# Autodesk Inventor assembly: ASY NDM_VOS pillar 1
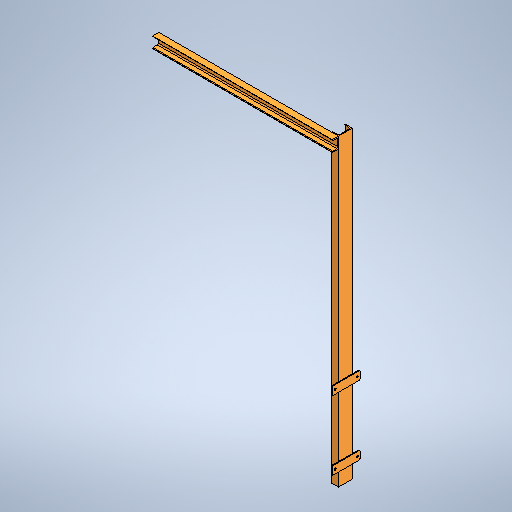
[picture p0: Inventor's stored thumbnail of the model, 512x512]
Saved by Autodesk Inventor 2025 (Build 290162010, 162A)
## iProperties
Created: 2025-11-03
Part Number: ASY NDM_VOS pillar 1
Document SubType Name: Assembly
Designer: admin
Mass: 33468.5 g
Surface Area: 12818.7 cm^2
Volume: 4385.61 cm^3
Density: 7.63143 g/cm^3
Author: admin
## Documents named in this file (5)
- C:\Users\admin\Yandex.Disk\home pc\Inventor\NDM-VOS_powder_hopper\400 tube\ASY NDM_VOS pillar 1.iam
- C:\Users\admin\Yandex.Disk\home pc\Inventor\NDM-VOS_powder_hopper\400 tube\NDM-VOS pillar 1 ch 1.ipt
- C:\Users\admin\Yandex.Disk\home pc\Inventor\NDM-VOS_powder_hopper\400 tube\Part2.ipt
- C:\Users\admin\Yandex.Disk\home pc\Inventor\NDM-VOS_powder_hopper\400 tube\NDM-VOS pillar 1 ch 2.ipt
- C:\Users\admin\Yandex.Disk\home pc\Inventor\NDM-VOS_powder_hopper\400 tube\NDM-VOS pillar 1 ch 3.ipt
## Components (6 placed, 4 different names)
1. NDM-VOS pillar 1 ch 1:1 — Mate:1, Mate:2, Rigid:2, Rigid:5, Rigid:6
2. Part2:1 — Flush:1, Rigid:5
3. NDM-VOS pillar 1 ch 2:1 — Rigid:2, Rigid:3, Rigid:4
4. Part2:2 — Rigid:3
5. NDM-VOS pillar 1 ch 3:1 — Rigid:4
6. Part2:3 — Rigid:6
## Relationships (8: WeldJoint 5, Mate 2, Flush 1)
- Mate:1: NDM-VOS pillar 1 ch 1:1
- Flush:1: Part2:1
- Mate:2: NDM-VOS pillar 1 ch 1:1
- Rigid:2 [WeldJoint]: NDM-VOS pillar 1 ch 1:1 ↔ NDM-VOS pillar 1 ch 2:1
- Rigid:3 [WeldJoint]: NDM-VOS pillar 1 ch 2:1 ↔ Part2:2
- Rigid:4 [WeldJoint]: NDM-VOS pillar 1 ch 2:1 ↔ NDM-VOS pillar 1 ch 3:1
- Rigid:5 [WeldJoint] (-100 mm): NDM-VOS pillar 1 ch 1:1 ↔ Part2:1
- Rigid:6 [WeldJoint] (-600 mm): NDM-VOS pillar 1 ch 1:1 ↔ Part2:3
